# Autodesk Inventor assembly: Main Assembly
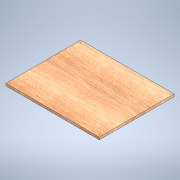
[picture p0: Inventor's stored thumbnail of the model, 180x180]
Saved by Autodesk Inventor 2020 (Build 240168000, 168)
## iProperties
Created: 2020-03-15
Part Number: Main Assembly
Document SubType Name: Assembly
Designer: Peter
Author: Peter
## Documents named in this file (3)
- C:\Users\Peter\Documents\Development\paragon-printer\Main Assembly.iam
- C:\Users\Peter\Documents\Development\paragon-printer\Stock\Base.ipt
- C:\Users\Peter\Documents\Development\paragon-printer\Paragon Printer Parameters.xlsx
## Components (1 placed, 1 different names)
1. Base:1
## Named parameters: base_x_dim = 500 mm, base_y_dim = 400 mm, base_thickness = 12.7 mm, twenty = 20 mm, tower_height = 300 mm
